# Autodesk Inventor assembly: Final assembly
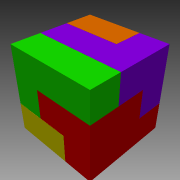
[picture p0: Inventor's stored thumbnail of the model, 180x180]
Saved by Autodesk Inventor 2013 (Build 170138000, 138)
## iProperties
Created: 2013-11-13
Part Number: Final assembly
Document SubType Name: Assembly
Designer: s601298
Author: s601298
## Documents named in this file (6)
- H:\IED7\Puzzle Cube\Final assembly.iam
- H:\IED7\Puzzle Cube\Part1.ipt
- H:\IED7\Puzzle Cube\Part2.ipt
- H:\IED7\Puzzle Cube\Part3.ipt
- H:\IED7\Puzzle Cube\Part4.ipt
- H:\IED7\Puzzle Cube\Part5.ipt
## Components (5 placed, 5 different names)
1. Part1:1 — Mate:1, Mate:2, Mate:3, Mate:4, Mate:11, Mate:13
2. Part2:1 — Mate:1, Mate:2, Mate:3, Mate:4, Mate:5, Mate:6, Mate:7, Mate:8, Mate:9, Mate:12
3. Part3:1 — Mate:5, Mate:6, Mate:7, Mate:10
4. Part4:1 — Mate:8, Mate:9, Mate:10
5. Part5:1 — Mate:11, Mate:12, Mate:13
## Relationships (13: Mate 13)
- Mate:1: Part1:1 ↔ Part2:1
- Mate:2: Part1:1 ↔ Part2:1
- Mate:3: Part1:1 ↔ Part2:1
- Mate:4: Part1:1 ↔ Part2:1
- Mate:5: Part2:1 ↔ Part3:1
- Mate:6: Part2:1 ↔ Part3:1
- Mate:7: Part2:1 ↔ Part3:1
- Mate:8: Part2:1 ↔ Part4:1
- Mate:9: Part2:1 ↔ Part4:1
- Mate:10: Part3:1 ↔ Part4:1
- Mate:11: Part1:1 ↔ Part5:1
- Mate:12: Part2:1 ↔ Part5:1
- Mate:13: Part1:1 ↔ Part5:1
